# Autodesk Inventor assembly: CrochetDeGrue
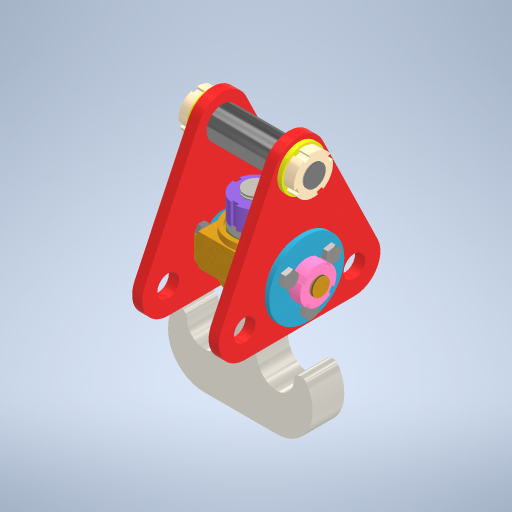
[picture p0: Inventor's stored thumbnail of the model, 512x512]
Saved by Autodesk Inventor 2023.2 (Build 272271030, 271C)
## iProperties
Created: 2023-03-30
Part Number: CrochetDeGrue
Document SubType Name: Assembly
Designer: Luis Valente
Author: Luis Valente
## Documents named in this file (13)
- C:\Users\lc010\OneDrive - Haute Ecole de Namur-Liege-Luxembourg\Henallux\Inventor School\Crochet de grue\CrochetDeGrue.iam
- C:\Users\lc010\OneDrive - Haute Ecole de Namur-Liege-Luxembourg\Henallux\Inventor School\Crochet de grue\1. CraneHook.ipt
- C:\Users\lc010\OneDrive - Haute Ecole de Namur-Liege-Luxembourg\Henallux\Inventor School\Crochet de grue\3. HookAnchor.ipt
- C:\Users\lc010\OneDrive - Haute Ecole de Namur-Liege-Luxembourg\Henallux\Inventor School\Crochet de grue\6. Bush.ipt
- C:\Users\lc010\OneDrive - Haute Ecole de Namur-Liege-Luxembourg\Henallux\Inventor School\Crochet de grue\2. SupportPlate.ipt
- C:\Users\lc010\OneDrive - Haute Ecole de Namur-Liege-Luxembourg\Henallux\Inventor School\Crochet de grue\4. EndBush.ipt
- C:\Users\lc010\OneDrive - Haute Ecole de Namur-Liege-Luxembourg\Henallux\Inventor School\Crochet de grue\7. LockNutM12.ipt
- C:\Users\lc010\OneDrive - Haute Ecole de Namur-Liege-Luxembourg\Henallux\Inventor School\Crochet de grue\10. Washer.ipt
- C:\Users\lc010\OneDrive - Haute Ecole de Namur-Liege-Luxembourg\Henallux\Inventor School\Crochet de grue\5. PlateSpacers.ipt
- C:\Users\lc010\OneDrive - Haute Ecole de Namur-Liege-Luxembourg\Henallux\Inventor School\Crochet de grue\8. LockNutM15.ipt
- C:\Users\lc010\OneDrive - Haute Ecole de Namur-Liege-Luxembourg\Henallux\Inventor School\Crochet de grue\9. LockNutM16.ipt
- C:\Users\lc010\OneDrive\Documentos\Inventor\Content Center Files\R2023\en-US\DIN 933\DIN 933 - M6  x 14.ipt
- C:\Users\lc010\OneDrive\Documentos\Inventor\Content Center Files\R2023\en-US\CSN EN 24 036\CSN EN 24 036 - M5.ipt
## Components (28 placed, 12 different names)
1. 1. CraneHook:1 — Rotational:1, Rotational:10
2. 3. HookAnchor:1 — Rotational:1, Rotational:2, Cylindrical:7, Cylindrical:8
3. 6. Bush:1 — Rotational:2, Rotational:9
4. 2. SupportPlate:1 — Cylindrical:7, Rotational:12, Rotational:3, Rotational:5, Insert:4, Insert:5, Insert:6
5. 2. SupportPlate:2 — Cylindrical:8, Rotational:14, Rotational:4, Rotational:6, Insert:10, Insert:11, Insert:12
6. 4. EndBush:1 — Rotational:12, Rotational:11, Insert:1, Insert:3
7. 4. EndBush:2 — Rotational:14, Rotational:13, Insert:7, Insert:8, Insert:9
8. 7. LockNutM12:1 — Rotational:11
9. 7. LockNutM12:2 — Rotational:13
10. 5. PlateSpacers:1 — Rotational:3, Rotational:4
11. 10. Washer:1 — Rotational:6, Rotational:7
12. 10. Washer:2 — Rotational:5, Rotational:8
13. 8. LockNutM15:1 — Rotational:7
14. 8. LockNutM15:2 — Rotational:8
15. 10. Washer:3 — Rotational:9
16. 9. LockNutM16:1 — Rotational:10
17. DIN 933 - replaced by DIN EN 24017 M6  x 14:1
18. DIN 933 - replaced by DIN EN 24017 M6  x 14:2 — Insert:1
19. DIN 933 - replaced by DIN EN 24017 M6  x 14:3 — Insert:3
20. CSN EN 24036 M5:1 — Insert:4
21. CSN EN 24036 M5:2 — Insert:5
22. CSN EN 24036 M5:3 — Insert:6
23. DIN 933 - replaced by DIN EN 24017 M6  x 14:4 — Insert:7
24. DIN 933 - replaced by DIN EN 24017 M6  x 14:5 — Insert:8
25. DIN 933 - replaced by DIN EN 24017 M6  x 14:6 — Insert:9
26. CSN EN 24036 M5:4 — Insert:10
27. CSN EN 24036 M5:5 — Insert:11
28. CSN EN 24036 M5:6 — Insert:12
## Relationships (29: RevoluteJoint 14, Insert 11, CylindricalJoint 2, Mate 2)
- Rotational:1 [RevoluteJoint]: 1. CraneHook:1 ↔ 3. HookAnchor:1
- Rotational:2 [RevoluteJoint]: 3. HookAnchor:1 ↔ 6. Bush:1
- Cylindrical:7: 3. HookAnchor:1 ↔ 2. SupportPlate:1
- Cylindrical:8: 3. HookAnchor:1 ↔ 2. SupportPlate:2
- Rotational:12 [RevoluteJoint]: 2. SupportPlate:1 ↔ 4. EndBush:1
- Rotational:14 [RevoluteJoint]: 2. SupportPlate:2 ↔ 4. EndBush:2
- Rotational:11 [RevoluteJoint]: 4. EndBush:1 ↔ 7. LockNutM12:1
- Rotational:13 [RevoluteJoint]: 4. EndBush:2 ↔ 7. LockNutM12:2
- Rotational:3 [RevoluteJoint]: 2. SupportPlate:1 ↔ 5. PlateSpacers:1
- Rotational:4 [RevoluteJoint]: 2. SupportPlate:2 ↔ 5. PlateSpacers:1
- Rotational:5 [RevoluteJoint]: 2. SupportPlate:1 ↔ 10. Washer:2
- Rotational:6 [RevoluteJoint]: 2. SupportPlate:2 ↔ 10. Washer:1
- Rotational:7 [RevoluteJoint]: 10. Washer:1 ↔ 8. LockNutM15:1
- Rotational:8 [RevoluteJoint]: 10. Washer:2 ↔ 8. LockNutM15:2
- Rotational:9 [RevoluteJoint]: 6. Bush:1 ↔ 10. Washer:3
- Rotational:10 [RevoluteJoint]: 1. CraneHook:1 ↔ 9. LockNutM16:1
- [Mate]: 4. EndBush:1 ↔ DIN 933 - replaced by DIN EN 24017 M6  x 14:1
- [Mate]: 4. EndBush:1 ↔ DIN 933 - replaced by DIN EN 24017 M6  x 14:1
- Insert:1: 4. EndBush:1 ↔ DIN 933 - replaced by DIN EN 24017 M6  x 14:2
- Insert:3: 4. EndBush:1 ↔ DIN 933 - replaced by DIN EN 24017 M6  x 14:3
- Insert:4: 2. SupportPlate:1 ↔ CSN EN 24036 M5:1
- Insert:5: 2. SupportPlate:1 ↔ CSN EN 24036 M5:2
- Insert:6: 2. SupportPlate:1 ↔ CSN EN 24036 M5:3
- Insert:7: 4. EndBush:2 ↔ DIN 933 - replaced by DIN EN 24017 M6  x 14:4
- Insert:8: 4. EndBush:2 ↔ DIN 933 - replaced by DIN EN 24017 M6  x 14:5
- Insert:9: 4. EndBush:2 ↔ DIN 933 - replaced by DIN EN 24017 M6  x 14:6
- Insert:10: 2. SupportPlate:2 ↔ CSN EN 24036 M5:4
- Insert:11: 2. SupportPlate:2 ↔ CSN EN 24036 M5:5
- Insert:12: 2. SupportPlate:2 ↔ CSN EN 24036 M5:6
